# Autodesk Inventor assembly: Assembly_KES400_Thorlabs_mounted
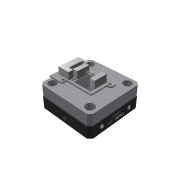
[picture p0: Inventor's stored thumbnail of the model, 180x180]
Saved by Autodesk Inventor 2019 (Build 230136000, 136)
## iProperties
Created: 2019-05-03
Part Number: Assembly_KES400_Thorlabs_mounted
Document SubType Name: Assembly
Designer: diederichbenedict
Author: diederichbenedict
## Documents named in this file (4)
- C:\Users\diederichbenedict\Dropbox\Dokumente\Promotion\PROJECTS\STORMoChip\INVENTOR\Nanoscopy-on-a-cheap\Assembly_KES400_Thorlabs_mounted.iam
- C:\Users\diederichbenedict\Dropbox\Dokumente\Promotion\PROJECTS\STORMoChip\INVENTOR\Nanoscopy-on-a-cheap\CP02_M-Step.ipt
- C:\Users\diederichbenedict\Dropbox\Dokumente\Promotion\PROJECTS\STORMoChip\INVENTOR\Nanoscopy-on-a-cheap\00_KES400.iam
- C:\Users\diederichbenedict\Dropbox\Dokumente\Promotion\PROJECTS\STORMoChip\INVENTOR\Nanoscopy-on-a-cheap\10_Adapter_KES400_Thorlabs.ipt
## Components (3 placed, 3 different names)
1. CP02_M-Step:1 — Insert:1, Angle:1, Flush:3
2. 00_KES400:1 [sub-assembly] — Insert:1, Angle:1, Flush:1, Flush:2
3. 10_Adapter_KES400_Thorlabs:1 — Flush:1, Flush:2, Flush:3
## Relationships (5: Flush 3, Insert 1, Angle 1)
- Insert:1 (10 mm): CP02_M-Step:1 ↔ 00_KES400:1
- Angle:1 (0 deg): CP02_M-Step:1 ↔ 00_KES400:1
- Flush:1: 00_KES400:1 ↔ 10_Adapter_KES400_Thorlabs:1
- Flush:2: 00_KES400:1 ↔ 10_Adapter_KES400_Thorlabs:1
- Flush:3: CP02_M-Step:1 ↔ 10_Adapter_KES400_Thorlabs:1
